# Autodesk Inventor assembly: main
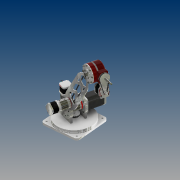
[picture p0: Inventor's stored thumbnail of the model, 180x180]
Saved by Autodesk Inventor 2020.3 (Build 243373000, 373)
## iProperties
Created: 2020-05-24
Part Number: main
Document SubType Name: Assembly
Designer: Svend
Author: Svend
## Documents named in this file (4)
- C:\Users\Svend\OneDrive\Documents\GitHub\BeerMinder\3D-model\boutjesEnMoertjes\main.iam
- C:\Users\Svend\OneDrive\Documents\GitHub\BeerMinder\3D-model\axis4\axis4.iam
- C:\Users\Svend\OneDrive\Documents\GitHub\BeerMinder\3D-model\axis3\axis3.iam
- C:\Users\Svend\OneDrive\Documents\GitHub\BeerMinder\3D-model\Base (Axis 1)\gefreesd\AssemblyGefreesdBasev2.iam
## Components (3 placed, 3 different names)
1. axis4:1 [sub-assembly] — Mate:5, Mate:6
2. axis3:1 [sub-assembly] — Mate:3, Mate:4, Mate:5, Mate:6
3. AssemblyGefreesdBasev2:1 [sub-assembly] — Mate:1, Mate:2, Flush:1, Mate:3, Mate:4
## Relationships (7: Mate 6, Flush 1)
- Mate:1: AssemblyGefreesdBasev2:1
- Mate:2: AssemblyGefreesdBasev2:1
- Flush:1: AssemblyGefreesdBasev2:1
- Mate:3: axis3:1 ↔ AssemblyGefreesdBasev2:1
- Mate:4: axis3:1 ↔ AssemblyGefreesdBasev2:1
- Mate:5: axis4:1 ↔ axis3:1
- Mate:6: axis4:1 ↔ axis3:1
